# Autodesk Inventor assembly: mascon-new
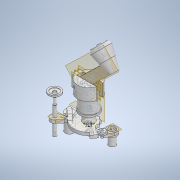
[picture p0: Inventor's stored thumbnail of the model, 180x180]
Saved by Autodesk Inventor 2022 (Build 260153000, 153)
## iProperties
Created: 2021-04-28
Part Number: mascon-new
Document SubType Name: Assembly
Designer: ben
Author: ben
## Documents named in this file (13)
- C:\Users\student\Desktop\r68-bve-mascon-test3\mascon-new.iam
- C:\Users\student\Desktop\r68-bve-mascon-test3\handle\handle.iam
- C:\Users\student\Desktop\r68-bve-mascon-test3\shell\shell.iam
- C:\Users\student\Desktop\r68-bve-mascon-test3\handle_base_rod.ipt
- C:\Users\student\Desktop\r68-bve-mascon-test3\handle_base_potholder.ipt
- C:\Users\student\Desktop\r68-bve-mascon-test3\handle_holder.ipt
- C:\Users\student\Desktop\r68-bve-mascon-test3\Reverser.ipt
- C:\Users\student\Desktop\r68-bve-mascon-test3\reverser-base.ipt
- C:\Users\student\Desktop\r68-bve-mascon-test3\NotchClickerAsm.iam
- C:\Users\student\Desktop\r68-bve-mascon-test3\ReverserNotch\ReverserClickAsm.iam
- C:\Users\student\Desktop\r68-bve-mascon-test3\handle-base\handle_base.iam
- C:\Users\student\Desktop\r68-bve-mascon-test3\handle_base2.ipt
- C:\Users\student\Desktop\r68-bve-mascon-test3\misc\V-wheel.ipt
## Components (12 placed, 12 different names)
1. shell:1 [sub-assembly] — Flush:4, Mate:14, Mate:15, Rotational:2, Flush:15, Mate:22
2. handle_base_rod:1 — Flush:11
3. handle_base_potholder:1 — Flush:9
4. handle_holder:1 — Mate:16
5. Reverser:1 — Flush:4, Flush:5
6. reverser-base:1 — Flush:5, Flush:6, Flush:10
7. NotchClickerAsm:1 [sub-assembly] — Mate:20, Mate:21, Flush:15, Mate:22
8. ReverserClickAsm:1 [sub-assembly] — Flush:14
9. handle:1 [sub-assembly] — Mate:17, Flush:12, Flush:13, Handle Pop
10. handle_base:1 [sub-assembly] — Mate:14, Mate:15, Mate:16, Mate:17, Rotational:2, Mate:18, Flush:8, Mate:19, Flush:11, Flush:12, Flush:13, Handle Pop
11. handle_base2:1 — Mate:18, Flush:8, Mate:19, Flush:9, Flush:14
12. V-wheel:1 — Mate:20, Mate:21
## Relationships (22: Flush 11, Mate 9, RevoluteJoint 2)
- Flush:4: shell:1 ↔ Reverser:1
- Flush:5: Reverser:1 ↔ reverser-base:1
- Flush:6 (-36.375 mm): reverser-base:1
- Mate:14: shell:1 ↔ handle_base:1
- Mate:15: shell:1 ↔ handle_base:1
- Mate:16: handle_holder:1 ↔ handle_base:1
- Mate:17: handle:1 ↔ handle_base:1
- Rotational:2 [RevoluteJoint] (-5 mm): shell:1 ↔ handle_base:1
- Mate:18: handle_base:1 ↔ handle_base2:1
- Flush:8: handle_base:1 ↔ handle_base2:1
- Mate:19: handle_base:1 ↔ handle_base2:1
- Flush:9: handle_base_potholder:1 ↔ handle_base2:1
- Mate:20: NotchClickerAsm:1 ↔ V-wheel:1
- Mate:21: NotchClickerAsm:1 ↔ V-wheel:1
- Flush:10: reverser-base:1
- Flush:11: handle_base_rod:1 ↔ handle_base:1
- Flush:12: handle:1 ↔ handle_base:1
- Flush:13: handle:1 ↔ handle_base:1
- Handle Pop [RevoluteJoint]: handle:1 ↔ handle_base:1
- Flush:14: ReverserClickAsm:1 ↔ handle_base2:1
- Flush:15: shell:1 ↔ NotchClickerAsm:1
- Mate:22: shell:1 ↔ NotchClickerAsm:1
